# Autodesk Inventor assembly: Drivetrain_Module
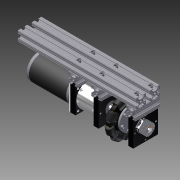
[picture p0: Inventor's stored thumbnail of the model, 180x180]
Saved by Autodesk Inventor 2012 (Build 160160000, 160)
## iProperties
Created: 2012-10-25
Part Number: Drivetrain_Module
Document SubType Name: Assembly
Designer: Andrew G. Meyer
Mass: 2167.83 g
Surface Area: 1864.84 cm^2
Volume: 699.231 cm^3
Density: 3.10031 g/cm^3
Author: Andrew G. Meyer
## Documents named in this file (12)
- C:\Users\Andrew G. Meyer\Documents\Projects\BallBot\macro\CAD\Drivetrain_Module.iam
- C:\Users\Andrew G. Meyer\Documents\Projects\BallBot\macro\CAD\P80\BB-56012.iam
- C:\Users\Andrew G. Meyer\Documents\Projects\BallBot\macro\CAD\wheel_key.ipt
- C:\Users\Andrew G. Meyer\Documents\Projects\BallBot\macro\CAD\500-key-hub\500-key-hub.ipt
- C:\Users\Andrew G. Meyer\Documents\Projects\BallBot\macro\CAD\Omni_Wheel\4-inch-omni-wheel.iam
- C:\Users\Andrew G. Meyer\Documents\Projects\BallBot\macro\CAD\BB25_block.iam
- C:\Users\Andrew G. Meyer\Documents\Inventor\Content Center Files\R2012\en-US\ANSI B18.3(05)\ANSI B18.3 - 10-32 UNF - 1(31).ipt
- C:\Users\Andrew G. Meyer\Documents\Inventor\Content Center Files\R2012\en-US\ANSI B18.6.3(36)\ANSI B18.6.3 - 10 - 32(2).ipt
- C:\Users\Andrew G. Meyer\Documents\Projects\BallBot\macro\CAD\AMT102-V\AMT102-V.ipt
- C:\Users\Andrew G. Meyer\Documents\Projects\BallBot\macro\CAD\drive_frame_spacer.iam
- C:\Users\Andrew G. Meyer\Documents\Projects\BallBot\macro\CAD\drive_frame_rail.iam
- C:\Users\Andrew G. Meyer\Documents\Inventor\Content Center Files\R2012\en-US\ANSI B18.3(05)\ANSI B18.3 - 1_4-20 UNC - 2.25(31).ipt
## Components (29 placed, 11 different names)
1. BB-56012:1 [sub-assembly] — Flush:1, Flush:2, Mate:4, Mate:5, Mate:6, Mate:8, Flush:4, Mate:9, Mate:13, Mate:14, Mate:15, Mate:16, Mate:17, Mate:18
2. wheel_key:1 — Mate:3, Flush:3, Mate:5, Mate:6
3. 500-key-hub:1 — Insert:1, Mate:3, Flush:3, Mate:4, Mate:7, Mate:8, Insert:2, Insert:3, Insert:4, Insert:5, Insert:6, Insert:7
4. 4-inch-omni-wheel:1 [sub-assembly] — Insert:1, Mate:7, Insert:8, Insert:9, Insert:10, Insert:11, Insert:12, Insert:13
5. BB25_block:1 [sub-assembly] — Flush:1, Flush:2, Flush:4, Flush:5, Angle:1, Mate:10, Mate:11, Mate:12
6. Hexagon Socket Head Cap Screw - Inch 10-32 UNF - 1:7 — Insert:6
7. Hexagon Socket Head Cap Screw - Inch 10-32 UNF - 1:8 — Insert:7
8. Hexagon Socket Head Cap Screw - Inch 10-32 UNF - 1:9 — Insert:4
9. Hexagon Socket Head Cap Screw - Inch 10-32 UNF - 1:10 — Insert:2
10. Hexagon Socket Head Cap Screw - Inch 10-32 UNF - 1:11 — Insert:3
11. Hexagon Socket Head Cap Screw - Inch 10-32 UNF - 1:12 — Insert:5
12. Hex Machine Screw Nut - Inch 10 - 32:7 — Insert:12
13. Hex Machine Screw Nut - Inch 10 - 32:8 — Insert:11
14. Hex Machine Screw Nut - Inch 10 - 32:9 — Insert:10
15. Hex Machine Screw Nut - Inch 10 - 32:10 — Insert:13
16. Hex Machine Screw Nut - Inch 10 - 32:11 — Insert:9
17. Hex Machine Screw Nut - Inch 10 - 32:12 — Insert:8
18. AMT102-V:1 — Flush:5, Mate:9, Angle:1
19. drive_frame_spacer:1 [sub-assembly] — Mate:16, Mate:17, Mate:18, Mate:21, Mate:22, Mate:25, Mate:26
20. drive_frame_spacer:2 [sub-assembly] — Mate:13, Mate:14, Mate:15, Mate:20, Mate:24
21. drive_frame_spacer:3 [sub-assembly] — Mate:10, Mate:11, Mate:12, Mate:19, Mate:23
22. drive_frame_rail:1 [sub-assembly] — Mate:23, Mate:24, Mate:25, Mate:26, Insert:15, Insert:17, Insert:19
23. drive_frame_rail:2 [sub-assembly] — Mate:19, Mate:20, Mate:21, Mate:22, Insert:14, Insert:16, Insert:18
24. Hexagon Socket Head Cap Screw - Inch 1/4 - 20 UNC - 2 1/4:7 — Insert:14
25. Hexagon Socket Head Cap Screw - Inch 1/4 - 20 UNC - 2 1/4:8 — Insert:15
26. Hexagon Socket Head Cap Screw - Inch 1/4 - 20 UNC - 2 1/4:9 — Insert:16
27. Hexagon Socket Head Cap Screw - Inch 1/4 - 20 UNC - 2 1/4:10 — Insert:18
28. Hexagon Socket Head Cap Screw - Inch 1/4 - 20 UNC - 2 1/4:11 — Insert:17
29. Hexagon Socket Head Cap Screw - Inch 1/4 - 20 UNC - 2 1/4:12 — Insert:19
## Relationships (49: Mate 24, Insert 19, Flush 5, Angle 1)
- Flush:1: BB-56012:1 ↔ BB25_block:1
- Flush:2: BB-56012:1 ↔ BB25_block:1
- Insert:1: 500-key-hub:1 ↔ 4-inch-omni-wheel:1
- Mate:3: wheel_key:1 ↔ 500-key-hub:1
- Flush:3: wheel_key:1 ↔ 500-key-hub:1
- Mate:4: BB-56012:1 ↔ 500-key-hub:1
- Mate:5: BB-56012:1 ↔ wheel_key:1
- Mate:6: BB-56012:1 ↔ wheel_key:1
- Mate:7: 500-key-hub:1 ↔ 4-inch-omni-wheel:1
- Mate:8 (25.4 mm): BB-56012:1 ↔ 500-key-hub:1
- Insert:2: 500-key-hub:1 ↔ Hexagon Socket Head Cap Screw - Inch 10-32 UNF - 1:10
- Insert:3: 500-key-hub:1 ↔ Hexagon Socket Head Cap Screw - Inch 10-32 UNF - 1:11
- Insert:4: 500-key-hub:1 ↔ Hexagon Socket Head Cap Screw - Inch 10-32 UNF - 1:9
- Insert:5: 500-key-hub:1 ↔ Hexagon Socket Head Cap Screw - Inch 10-32 UNF - 1:12
- Insert:6: 500-key-hub:1 ↔ Hexagon Socket Head Cap Screw - Inch 10-32 UNF - 1:7
- Insert:7: 500-key-hub:1 ↔ Hexagon Socket Head Cap Screw - Inch 10-32 UNF - 1:8
- Insert:8: 4-inch-omni-wheel:1 ↔ Hex Machine Screw Nut - Inch 10 - 32:12
- Insert:9: 4-inch-omni-wheel:1 ↔ Hex Machine Screw Nut - Inch 10 - 32:11
- Insert:10: 4-inch-omni-wheel:1 ↔ Hex Machine Screw Nut - Inch 10 - 32:9
- Insert:11: 4-inch-omni-wheel:1 ↔ Hex Machine Screw Nut - Inch 10 - 32:8
- Insert:12: 4-inch-omni-wheel:1 ↔ Hex Machine Screw Nut - Inch 10 - 32:7
- Insert:13: 4-inch-omni-wheel:1 ↔ Hex Machine Screw Nut - Inch 10 - 32:10
- Flush:4: BB-56012:1 ↔ BB25_block:1
- Flush:5: BB25_block:1 ↔ AMT102-V:1
- Mate:9: BB-56012:1 ↔ AMT102-V:1
- Angle:1 (45 deg): BB25_block:1 ↔ AMT102-V:1
- Mate:10: BB25_block:1 ↔ drive_frame_spacer:3
- Mate:11: BB25_block:1 ↔ drive_frame_spacer:3
- Mate:12: BB25_block:1 ↔ drive_frame_spacer:3
- Mate:13: BB-56012:1 ↔ drive_frame_spacer:2
- Mate:14: BB-56012:1 ↔ drive_frame_spacer:2
- Mate:15: BB-56012:1 ↔ drive_frame_spacer:2
- Mate:16: BB-56012:1 ↔ drive_frame_spacer:1
- Mate:17: BB-56012:1 ↔ drive_frame_spacer:1
- Mate:18: BB-56012:1 ↔ drive_frame_spacer:1
- Mate:19: drive_frame_spacer:3 ↔ drive_frame_rail:2
- Mate:20: drive_frame_spacer:2 ↔ drive_frame_rail:2
- Mate:21: drive_frame_spacer:1 ↔ drive_frame_rail:2
- Mate:22: drive_frame_spacer:1 ↔ drive_frame_rail:2
- Mate:23: drive_frame_spacer:3 ↔ drive_frame_rail:1
- Mate:24: drive_frame_spacer:2 ↔ drive_frame_rail:1
- Mate:25: drive_frame_spacer:1 ↔ drive_frame_rail:1
- Mate:26: drive_frame_spacer:1 ↔ drive_frame_rail:1
- Insert:14: drive_frame_rail:2 ↔ Hexagon Socket Head Cap Screw - Inch 1/4 - 20 UNC - 2 1/4:7
- Insert:15: drive_frame_rail:1 ↔ Hexagon Socket Head Cap Screw - Inch 1/4 - 20 UNC - 2 1/4:8
- Insert:16: drive_frame_rail:2 ↔ Hexagon Socket Head Cap Screw - Inch 1/4 - 20 UNC - 2 1/4:9
- Insert:17: drive_frame_rail:1 ↔ Hexagon Socket Head Cap Screw - Inch 1/4 - 20 UNC - 2 1/4:11
- Insert:18: drive_frame_rail:2 ↔ Hexagon Socket Head Cap Screw - Inch 1/4 - 20 UNC - 2 1/4:10
- Insert:19: drive_frame_rail:1 ↔ Hexagon Socket Head Cap Screw - Inch 1/4 - 20 UNC - 2 1/4:12
